# Autodesk Inventor assembly: fc17-064
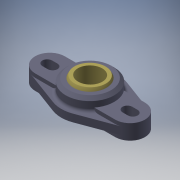
[picture p0: Inventor's stored thumbnail of the model, 180x180]
Saved by Autodesk Inventor 2017.1 (Build 211199000, 199)
## iProperties
Category: Bearing
Company: Autodesk, Inc.
Created: 2016-12-16
Part Number: fc17-064
Document SubType Name: Assembly
Project: FIRST
Catalog Web Link: http://www.igus.com/wpck/5378/igubal_Flanschlager_EFOI?C=US&L=en
Description: Flanged spherical bearing
Vendor: igus
Engineer: Autodesk, Inc.
Title: Flanged Spherical Bearing
Author: Autodesk, Inc.
Keywords: FIRST Choice
## Documents named in this file (3)
- D:\FIRST\FIRST KOP 2017\FIRST FirstChoice 2017\fc17-064_Bearing.iam
- D:\FIRST\FIRST KOP 2017\FIRST FirstChoice 2017\Parts\EFOI-10_Housing.ipt
- D:\FIRST\FIRST KOP 2017\FIRST FirstChoice 2017\Parts\EFOI-10_Spherical Bearing.ipt
## Components (2 placed, 2 different names)
1. EFOI-10_Housing:1 — Mate:1
2. EFOI-10_Spherical Bearing:1 — Mate:1
## Relationships (1: Mate 1)
- Mate:1: EFOI-10_Housing:1 ↔ EFOI-10_Spherical Bearing:1
